# Autodesk Inventor assembly: BIC Round Stic Pen Assembly
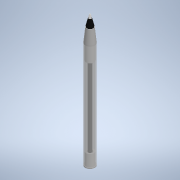
[picture p0: Inventor's stored thumbnail of the model, 180x180]
Saved by Autodesk Inventor 2021 (Build 250183000, 183)
## iProperties
Created: 2020-03-16
Part Number: BIC Round Stic Pen Assembly
Document SubType Name: Assembly
Designer: Daniel
Author: Daniel
## Documents named in this file (5)
- F:\bic-round-stic-pen-2.snapshot.15\Inventor\BIC Round Stic Pen Assembly.iam
- F:\bic-round-stic-pen-2.snapshot.15\Inventor\Barrel.ipt
- F:\bic-round-stic-pen-2.snapshot.15\Inventor\Barrel End Cap.ipt
- F:\bic-round-stic-pen-2.snapshot.15\Inventor\Barrel to Tip Stopper.ipt
- F:\bic-round-stic-pen-2.snapshot.15\Inventor\Ink Barrel + Tip.ipt
## Components (4 placed, 4 different names)
1. Barrel:1 — Rotational:1, Rotational:2
2. Barrel End Cap:1 — Rotational:1
3. Barrel to Tip Stopper:1 — Rotational:2, Rotational:3
4. Ink Barrel + Tip:1 — Rotational:3
## Relationships (3: RevoluteJoint 3)
- Rotational:1 [RevoluteJoint]: Barrel:1 ↔ Barrel End Cap:1
- Rotational:2 [RevoluteJoint]: Barrel:1 ↔ Barrel to Tip Stopper:1
- Rotational:3 [RevoluteJoint]: Barrel to Tip Stopper:1 ↔ Ink Barrel + Tip:1
